# Autodesk Inventor assembly: Assembly shaft 1 sprocect
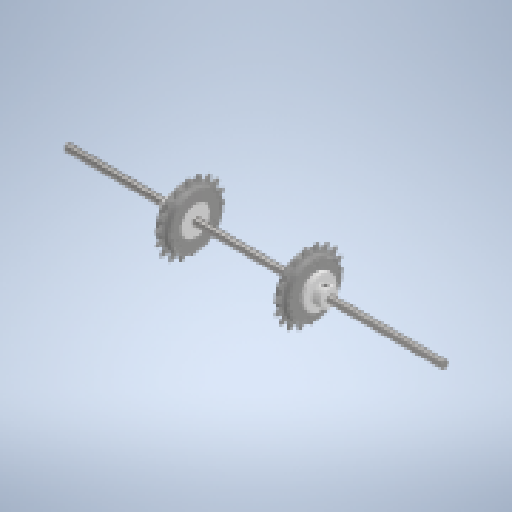
[picture p0: Inventor's stored thumbnail of the model, 512x512]
Saved by Autodesk Inventor 2026.1 (Build 301233020, 233B)
## iProperties
Created: 2026-01-23
Part Number: Assembly shaft 1 sprocect
Document SubType Name: Assembly
Designer: user
Author: user
## Documents named in this file (4)
- D:\asu\machine element design\project\design - Copy\Assembly shaft 1 sprocect.iam
- D:\asu\machine element design\project\design - Copy\shaft.ipt
- D:\asu\machine element design\project\design - Copy\18t_single-speed_freewheel-1.snapshot.1\18T_ss_fw\18T_ss_fw\18T_ss_fw.iam
- D:\asu\machine element design\project\design - Copy\sprocet adaptor.ipt
## Components (5 placed, 3 different names)
1. shaft:1 — Mate:3, Mate:6, Mate:7, Mate:8
2. 18T_ss_fw:1 [sub-assembly] — Mate:1, Mate:2, Mate:8
3. 18T_ss_fw:2 [sub-assembly] — Mate:4, Mate:5, Mate:6, Mate:7
4. sprocet adaptor:1 — Mate:4, Mate:5
5. sprocet adaptor:2 — Mate:1, Mate:2, Mate:3
## Relationships (8: Mate 8)
- Mate:1: 18T_ss_fw:1 ↔ sprocet adaptor:2
- Mate:2: 18T_ss_fw:1 ↔ sprocet adaptor:2
- Mate:3: shaft:1 ↔ sprocet adaptor:2
- Mate:4: 18T_ss_fw:2 ↔ sprocet adaptor:1
- Mate:5: 18T_ss_fw:2 ↔ sprocet adaptor:1
- Mate:6: shaft:1 ↔ 18T_ss_fw:2
- Mate:7 (-140 mm): shaft:1 ↔ 18T_ss_fw:2
- Mate:8 (-140 mm): shaft:1 ↔ 18T_ss_fw:1
